# Autodesk Inventor assembly: SESTAVA PLOCHA S DRŽÁKEM MOTOTŮ
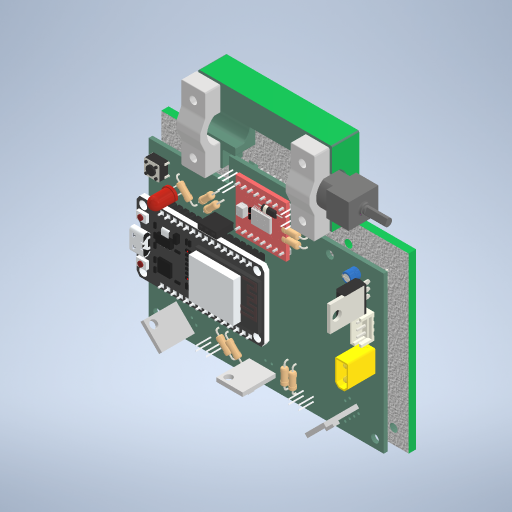
[picture p0: Inventor's stored thumbnail of the model, 512x512]
Saved by Autodesk Inventor 2024 (Build 280153000, 153)
## iProperties
Created: 2023-08-14
Part Number: SESTAVA PLOCHA S DRŽÁKEM MOTOTŮ
Document SubType Name: Assembly
Designer: jaryj
Author: jaryj
## Documents named in this file (5)
- C:\Users\jaryj\Desktop\Škola\Mini sumo\RoboCop\- 3D -\temporary\SESTAVA PLOCHA S DRŽÁKEM MOTOTŮ.iam
- C:\Users\jaryj\Desktop\Škola\Mini sumo\RoboCop\- 3D -\temporary\sumec plocha s držákem motorů.ipt
- C:\Users\jaryj\Desktop\Škola\Mini sumo\RoboCop\- 3D -\temporary\Objímka motoru pro plochu s držákem.ipt
- C:\Users\jaryj\Desktop\Škola\Mini sumo\RoboCop\- PCB -\sumec\sumec.iam
- C:\Users\jaryj\Desktop\Škola\Mini sumo\RoboCop\- 3D -\archive\pcb_1.0\GA12-N20_Motor.ipt
## Components (5 placed, 4 different names)
1. sumec plocha s držákem motorů:1 — Tuhé:1, Tuhé:2, Tuhé:3, Proti sobě:1, Stejný směr:1, Tečnost:1
2. Objímka motoru pro plochu s držákem:1 — Tuhé:3
3. Objímka motoru pro plochu s držákem:2 — Tuhé:2
4. sumec:1 [sub-assembly] — Tuhé:1
5. GA12-N20_Motor:1 — Proti sobě:1, Stejný směr:1, Tečnost:1
## Relationships (6: WeldJoint 3, Mate 1, Flush 1, Tangent 1)
- Tuhé:1 [WeldJoint] (-6 mm): sumec plocha s držákem motorů:1 ↔ sumec:1
- Tuhé:2 [WeldJoint] (-1 mm): sumec plocha s držákem motorů:1 ↔ Objímka motoru pro plochu s držákem:2
- Tuhé:3 [WeldJoint] (-1 mm): sumec plocha s držákem motorů:1 ↔ Objímka motoru pro plochu s držákem:1
- Proti sobě:1 [Mate] (0.125 mm): sumec plocha s držákem motorů:1 ↔ GA12-N20_Motor:1
- Stejný směr:1 [Flush]: sumec plocha s držákem motorů:1 ↔ GA12-N20_Motor:1
- Tečnost:1 [Tangent] (0.125 mm): sumec plocha s držákem motorů:1 ↔ GA12-N20_Motor:1
